# Autodesk Inventor assembly: PistaoEquipado
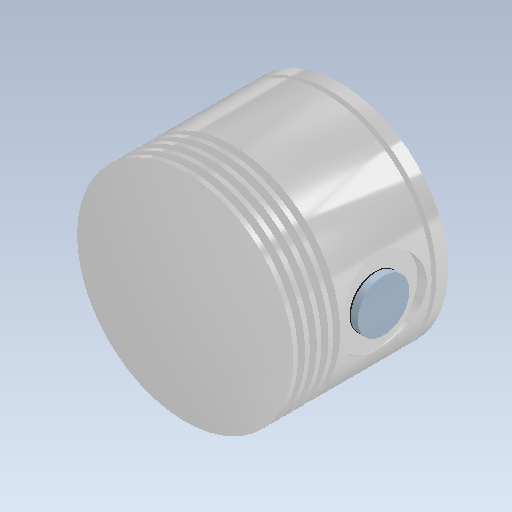
[picture p0: Inventor's stored thumbnail of the model, 512x512]
Saved by Autodesk Inventor 2021 (Build 250183000, 183)
## iProperties
Created: 2021-07-24
Part Number: PistaoEquipado
Document SubType Name: Assembly
Designer: Giovanni
Author: Giovanni
## Documents named in this file (4)
- C:\Users\irineu\Documents\Inventor\MotorRadial7\PistaoEquipado.iam
- C:\Users\irineu\Documents\Inventor\MotorRadial7\Pistão.ipt
- C:\Users\irineu\Documents\Inventor\MotorRadial7\Pino do Pistão.ipt
- C:\Users\irineu\Documents\Inventor\MotorRadial7\Plug do Pistão.ipt
## Components (4 placed, 3 different names)
1. Pistão:1 — Alinhado:1, Alinhado:2, Coincidente:1, Coincidente:2
2. Pino do Pistão:1 — Coincidente:2, Coincidente:3, Inserir:1, Inserir:2
3. Plug do Pistão:1 — Inserir:2
4. Plug do Pistão:2 — Inserir:1
## Relationships (7: Mate 3, Flush 2, Insert 2)
- Alinhado:1 [Flush]: Pistão:1
- Alinhado:2 [Flush]: Pistão:1
- Coincidente:1 [Mate]: Pistão:1
- Coincidente:2 [Mate]: Pistão:1 ↔ Pino do Pistão:1
- Coincidente:3 [Mate]: Pino do Pistão:1
- Inserir:1: Pino do Pistão:1 ↔ Plug do Pistão:2
- Inserir:2: Pino do Pistão:1 ↔ Plug do Pistão:1
